# Autodesk Inventor assembly: Body Cover Assembly
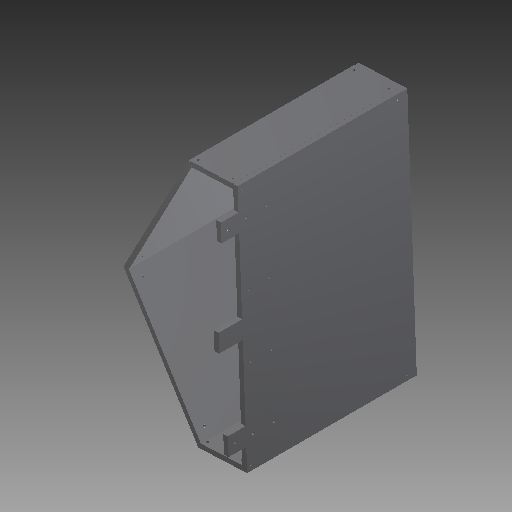
[picture p0: Inventor's stored thumbnail of the model, 512x512]
Saved by Autodesk Inventor 2017 (Build 210142000, 142)
## iProperties
Created: 2018-10-18
Part Number: Body Cover Assembly
Document SubType Name: Assembly
Designer: Dell
Author: Dell
## Documents named in this file (5)
- C:\Users\Dell\Documents\GitHub\tr2\Body\Body Cover Assembly.iam
- C:\Users\Dell\Documents\GitHub\tr2\Body\BO07.ipt
- C:\Users\Dell\Documents\GitHub\tr2\Body\BO08.ipt
- C:\Users\Dell\Documents\GitHub\tr2\Body\BO10.ipt
- C:\Users\Dell\Documents\GitHub\tr2\Body\BO11.ipt
## Components (6 placed, 4 different names)
1. BO07:1 — Flush:4, Mate:20, Mate:32
2. BO08:2 — Mate:29, Flush:6, Mate:32, Mate:33
3. BO08:3 — Mate:19, Flush:5, Mate:34, Flush:7
4. BO07:2 — Mate:19, Flush:4, Mate:20, Flush:5, Mate:36
5. BO10:1 — Mate:29, Flush:6, Mate:33, Mate:34, Flush:7, Mate:35, Flush:8
6. BO11:2 — Mate:35, Mate:36, Flush:8
## Relationships (13: Mate 8, Flush 5)
- Mate:19: BO08:3 ↔ BO07:2
- Flush:4: BO07:1 ↔ BO07:2
- Mate:20: BO07:1 ↔ BO07:2
- Flush:5: BO08:3 ↔ BO07:2
- Mate:29: BO08:2 ↔ BO10:1
- Flush:6: BO08:2 ↔ BO10:1
- Mate:32: BO07:1 ↔ BO08:2
- Mate:33: BO08:2 ↔ BO10:1
- Mate:34: BO08:3 ↔ BO10:1
- Flush:7: BO08:3 ↔ BO10:1
- Mate:35: BO10:1 ↔ BO11:2
- Mate:36: BO07:2 ↔ BO11:2
- Flush:8: BO10:1 ↔ BO11:2
